# Autodesk Inventor assembly: Piston
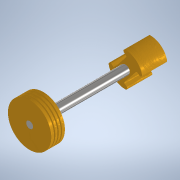
[picture p0: Inventor's stored thumbnail of the model, 180x180]
Saved by Autodesk Inventor 2020 (Build 240168000, 168)
## iProperties
Created: 2021-10-28
Part Number: Piston
Document SubType Name: Assembly
Designer: simon.erikssonwestl
Author: simon.erikssonwestl
## Documents named in this file (4)
- C:\Users\simon.erikssonwestl\Documents\Inventor\Ång\Assemblies\Piston.iam
- C:\Users\simon.erikssonwestl\Documents\Inventor\Ång\Part29.ipt
- C:\Users\simon.erikssonwestl\Documents\Inventor\Ång\Part28.ipt
- C:\Users\simon.erikssonwestl\Documents\Inventor\Ång\Part30.ipt
## Components (3 placed, 3 different names)
1. Part29:1 — Mate:1, Mate:4
2. Part28:1 — Mate:1, Mate:2, Mate:3, Mate:4
3. Part30:1 — Mate:2, Mate:3
## Relationships (4: Mate 4)
- Mate:1: Part29:1 ↔ Part28:1
- Mate:2: Part28:1 ↔ Part30:1
- Mate:3: Part28:1 ↔ Part30:1
- Mate:4: Part29:1 ↔ Part28:1
